# Autodesk Inventor assembly: calas_montaña
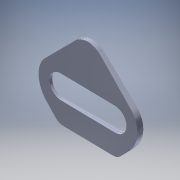
[picture p0: Inventor's stored thumbnail of the model, 180x180]
Saved by Autodesk Inventor 2019 (Build 230136000, 136)
## iProperties
Created: 2019-01-30
Part Number: calas_montaña
Document SubType Name: Assembly
Designer: assman
Author: assman
## Documents named in this file (2)
- D:\Inventor\Projects\Calas Montaña\calas_montaña.iam
- D:\Inventor\STL\SPD_Cleat_Wedge.ipt
## Components (2 placed, 1 different names)
1. SPD_Cleat_Wedge:1 — Rigid:1
2. SPD_Cleat_Wedge:2 — Rigid:1
## Relationships (1: WeldJoint 1)
- Rigid:1 [WeldJoint]: SPD_Cleat_Wedge:1 ↔ SPD_Cleat_Wedge:2
